# Autodesk Inventor assembly: BOX_WOOD
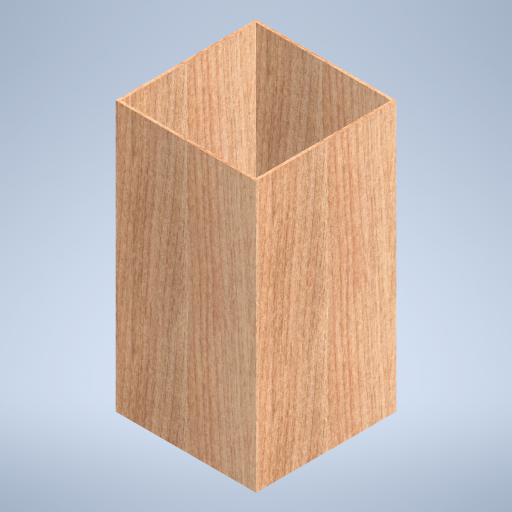
[picture p0: Inventor's stored thumbnail of the model, 512x512]
Saved by Autodesk Inventor 2023 (Build 270158000, 158)
## iProperties
Created: 2024-02-10
Part Number: BOX_WOOD
Document SubType Name: Assembly
Designer: vraco
Author: vraco
## Documents named in this file (5)
- C:\Users\vraco\Documents\Inventor\kos_e-cigarety\BOX_WOOD.iam
- C:\Users\vraco\Documents\Inventor\kos_e-cigarety\BOTTOM_PART_BOX.ipt
- C:\Users\vraco\Documents\Inventor\kos_e-cigarety\SIDE_PART_BOX.ipt
- C:\Users\vraco\Documents\Inventor\kos_e-cigarety\DISTANCE_BRICK_BOTTOM.ipt
- C:\Users\vraco\Documents\Inventor\kos_e-cigarety\DISTANCE_BRICK_SIDE.ipt
## Components (13 placed, 5 different names)
1. BOTTOM_PART_BOX:1 — Flush:1, Mate:1, Mate:2, Mate:3, Mate:7, Mate:8, Flush:7, Flush:8, Flush:9, Flush:10, Flush:11, Flush:12, Flush:13, Flush:14, Flush:15, Flush:16, Flush:18, Mate:12, Flush:20, Mate:13, Flush:22, Mate:14, Flush:24, Mate:15, Mate:16, Mate:17
2. 1 — Mate:1, Flush:2, Mate:2, Mate:4
3. SIDE_PART_BOX:3 — Flush:3, Mate:3, Mate:4
4. SIDE_PART_BOX:5 — Flush:5, Mate:7, Mate:9, Flush:17, Flush:19, Flush:21, Flush:23
5. SIDE_PART_BOX:6 — Flush:6, Mate:8, Mate:9
6. DISTANCE_BRICK_BOTTOM:1 — Flush:7, Flush:8, Flush:9, Mate:11
7. DISTANCE_BRICK_BOTTOM:2 — Flush:10, Flush:11, Flush:12, Mate:10
8. DISTANCE_BRICK_BOTTOM:3 — Flush:13, Flush:14, Mate:10
9. DISTANCE_BRICK_BOTTOM:4 — Flush:15, Flush:16, Mate:11
10. DISTANCE_BRICK_SIDE:1 — Flush:17, Flush:18, Mate:12
11. DISTANCE_BRICK_SIDE:2 — Flush:19, Flush:20, Mate:13
12. DISTANCE_BRICK_SIDE:3 — Flush:21, Flush:22, Mate:14
13. DISTANCE_BRICK_SIDE:4 — Flush:23, Flush:24, Mate:15
## Relationships (38: Flush 23, Mate 15)
- Flush:1: BOTTOM_PART_BOX:1
- Mate:1: BOTTOM_PART_BOX:1 ↔ 1
- Flush:2: 1
- Mate:2: BOTTOM_PART_BOX:1 ↔ 1
- Flush:3: SIDE_PART_BOX:3
- Mate:3: BOTTOM_PART_BOX:1 ↔ SIDE_PART_BOX:3
- Mate:4: 1 ↔ SIDE_PART_BOX:3
- Flush:5: SIDE_PART_BOX:5
- Mate:7: BOTTOM_PART_BOX:1 ↔ SIDE_PART_BOX:5
- Flush:6: SIDE_PART_BOX:6
- Mate:8: BOTTOM_PART_BOX:1 ↔ SIDE_PART_BOX:6
- Mate:9: SIDE_PART_BOX:5 ↔ SIDE_PART_BOX:6
- Flush:7: BOTTOM_PART_BOX:1 ↔ DISTANCE_BRICK_BOTTOM:1
- Flush:8: BOTTOM_PART_BOX:1 ↔ DISTANCE_BRICK_BOTTOM:1
- Flush:9: BOTTOM_PART_BOX:1 ↔ DISTANCE_BRICK_BOTTOM:1
- Flush:10: BOTTOM_PART_BOX:1 ↔ DISTANCE_BRICK_BOTTOM:2
- Flush:11: BOTTOM_PART_BOX:1 ↔ DISTANCE_BRICK_BOTTOM:2
- Flush:12: BOTTOM_PART_BOX:1 ↔ DISTANCE_BRICK_BOTTOM:2
- Flush:13: BOTTOM_PART_BOX:1 ↔ DISTANCE_BRICK_BOTTOM:3
- Flush:14: BOTTOM_PART_BOX:1 ↔ DISTANCE_BRICK_BOTTOM:3
- Mate:10 (90 mm): DISTANCE_BRICK_BOTTOM:2 ↔ DISTANCE_BRICK_BOTTOM:3
- Flush:15: BOTTOM_PART_BOX:1 ↔ DISTANCE_BRICK_BOTTOM:4
- Flush:16: BOTTOM_PART_BOX:1 ↔ DISTANCE_BRICK_BOTTOM:4
- Mate:11 (90 mm): DISTANCE_BRICK_BOTTOM:1 ↔ DISTANCE_BRICK_BOTTOM:4
- Flush:17: SIDE_PART_BOX:5 ↔ DISTANCE_BRICK_SIDE:1
- Flush:18: BOTTOM_PART_BOX:1 ↔ DISTANCE_BRICK_SIDE:1
- Mate:12 (30 mm): BOTTOM_PART_BOX:1 ↔ DISTANCE_BRICK_SIDE:1
- Flush:19: SIDE_PART_BOX:5 ↔ DISTANCE_BRICK_SIDE:2
- Flush:20: BOTTOM_PART_BOX:1 ↔ DISTANCE_BRICK_SIDE:2
- Mate:13 (30 mm): BOTTOM_PART_BOX:1 ↔ DISTANCE_BRICK_SIDE:2
- Flush:21: SIDE_PART_BOX:5 ↔ DISTANCE_BRICK_SIDE:3
- Flush:22: BOTTOM_PART_BOX:1 ↔ DISTANCE_BRICK_SIDE:3
- Mate:14 (250 mm): BOTTOM_PART_BOX:1 ↔ DISTANCE_BRICK_SIDE:3
- Flush:23: SIDE_PART_BOX:5 ↔ DISTANCE_BRICK_SIDE:4
- Flush:24: BOTTOM_PART_BOX:1 ↔ DISTANCE_BRICK_SIDE:4
- Mate:15 (250 mm): BOTTOM_PART_BOX:1 ↔ DISTANCE_BRICK_SIDE:4
- Mate:16: BOTTOM_PART_BOX:1
- Mate:17: BOTTOM_PART_BOX:1
